# Autodesk Inventor assembly: Assembly1
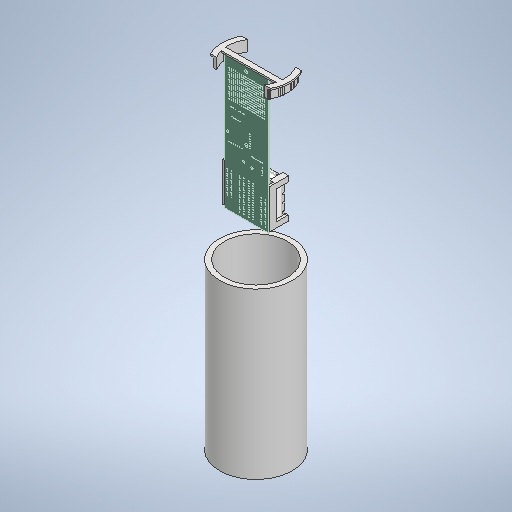
[picture p0: Inventor's stored thumbnail of the model, 512x512]
Saved by Autodesk Inventor 2025 (Build 290162010, 162A)
## iProperties
Created: 2024-07-03
Part Number: Assembly1
Document SubType Name: Assembly
Designer: vncnt
Author: vncnt
## Documents named in this file (6)
- C:\Users\vncnt\Documents\GitHub\Air-Quality-Sensor\M_CAD-Inventor\Assembly1.iam
- C:\Users\vncnt\Documents\GitHub\Air-Quality-Sensor\M_CAD-Inventor\PVC.ipt
- C:\Users\vncnt\Documents\GitHub\Air-Quality-Sensor\M_CAD-Inventor\CSL_AQS_V1_spin3.iam
- C:\Users\vncnt\Documents\GitHub\Air-Quality-Sensor\M_CAD-Inventor\AQS_Mount.ipt
- C:\Users\vncnt\Documents\GitHub\Air-Quality-Sensor\M_CAD-Inventor\SEN5X_Mount.ipt
- C:\Users\vncnt\Documents\GitHub\Air-Quality-Sensor\M_CAD-Inventor\Sensirion_STEP_SEN5x\Sensirion_STEP_SEN5x.ipt
## Components (5 placed, 5 different names)
1. PVC:1 — Mate:1, Mate:2, Flush:1
2. CSL_AQS_V1_spin3:1 [sub-assembly] — Mate:3, Mate:4, Mate:5, Flush:2, Angle:1
3. AQS_Mount:1 — Mate:1, Mate:2, Flush:1, Mate:3, Mate:4
4. SEN5X_Mount:1 — Mate:5, Flush:2, Angle:1, Mate:6, Mate:7, Mate:8
5. Sensirion_STEP_SEN5x:1 — Mate:6, Mate:7, Mate:8
## Relationships (11: Mate 8, Flush 2, Angle 1)
- Mate:1: PVC:1 ↔ AQS_Mount:1
- Mate:2: PVC:1 ↔ AQS_Mount:1
- Flush:1: PVC:1 ↔ AQS_Mount:1
- Mate:3: CSL_AQS_V1_spin3:1 ↔ AQS_Mount:1
- Mate:4: CSL_AQS_V1_spin3:1 ↔ AQS_Mount:1
- Mate:5: CSL_AQS_V1_spin3:1 ↔ SEN5X_Mount:1
- Flush:2: CSL_AQS_V1_spin3:1 ↔ SEN5X_Mount:1
- Angle:1 (270 deg): CSL_AQS_V1_spin3:1 ↔ SEN5X_Mount:1
- Mate:6: SEN5X_Mount:1 ↔ Sensirion_STEP_SEN5x:1
- Mate:7: SEN5X_Mount:1 ↔ Sensirion_STEP_SEN5x:1
- Mate:8: SEN5X_Mount:1 ↔ Sensirion_STEP_SEN5x:1
